# Autodesk Inventor assembly: Funnel Right
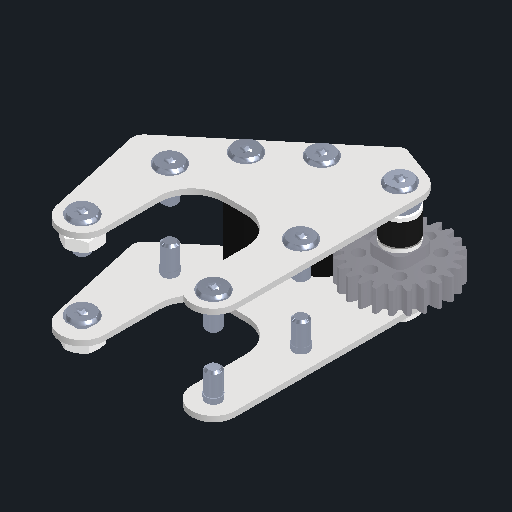
[picture p0: Inventor's stored thumbnail of the model, 512x512]
Saved by Autodesk Inventor 2025 (Build 290162000, 162)
## iProperties
Created: 2024-10-18
Part Number: Funnel Right
Document SubType Name: Assembly
Designer: Averey Ku
Author: averey
## Documents named in this file (19)
- D:\VEX\High Stakes\CAD\V2\Chassis\Drivebay Right\Funnel Right.iam
- D:\VEX\High Stakes\CAD\V2\Chassis\Drivebay Right\Funnel Gusset Right.ipt
- D:\VEX\High Stakes\CAD\ROBOPROS-CAD-Inventor\Motion\Spacers\Spacer Nylon .375 OD\NSpacer .375 OD x .500.ipt
- D:\VEX\High Stakes\CAD\ROBOPROS-CAD-Inventor\Motion\Spacers\Spacer Nylon .375 OD.ipt
- D:\VEX\High Stakes\CAD\ROBOPROS-CAD-Inventor\Structure\Hardware\Screw Steel - Star\SScrew Star Smooth 1.250.ipt
- D:\VEX\High Stakes\CAD\ROBOPROS-CAD-Inventor\Structure\Hardware\Screw Steel - Star.ipt
- D:\VEX\High Stakes\CAD\ROBOPROS-CAD-Inventor\Structure\Hardware\Nut Nylon\Nut Nylon - White.ipt
- D:\VEX\High Stakes\CAD\ROBOPROS-CAD-Inventor\Structure\Hardware\Nut Nylon.ipt
- D:\VEX\High Stakes\CAD\ROBOPROS-CAD-Inventor\Structure\Hardware\Screw Shoulder Robosource\SScrew Shoulder Smooth .375 x .12.ipt
- D:\VEX\High Stakes\CAD\ROBOPROS-CAD-Inventor\Structure\Hardware\Screw Shoulder Robosource.ipt
- D:\VEX\High Stakes\CAD\V2\Chassis\Drivebay Right\Half Cut HS 24T Gear, No Insert Right.ipt
- D:\VEX\High Stakes\CAD\V2\Chassis\Drivebay Right\Nut Keps Right1.ipt
- D:\vex_robotics_high_stakes\hardware\cad\VEX-CAD-Inventor\Motion\Spacers\Spacer Nylon .375 OD\NSpacer .375 OD x .250.ipt
- D:\vex_robotics_high_stakes\hardware\cad\VEX-CAD-Inventor\Motion\Spacers\Spacer Nylon .375 OD.ipt
- D:\vex_robotics_high_stakes\hardware\cad\VEX-CAD-Inventor\Motion\Spacers\Washer Teflon\TWasher .375 OD x .04000.ipt
- D:\vex_robotics_high_stakes\hardware\cad\VEX-CAD-Inventor\Motion\Spacers\Washer Teflon.ipt
- D:\vex_robotics_high_stakes\hardware\cad\VEX-CAD-Inventor\Motion\Spacers\Washer Steel\SWasher .375 OD x .015625.ipt
- D:\vex_robotics_high_stakes\hardware\cad\VEX-CAD-Inventor\Motion\Spacers\Washer Steel.ipt
- D:\VEX\High Stakes\CAD\ROBOPROS-CAD-Inventor\Structure\Hardware\Screw Shoulder Robosource\SScrew Shoulder Smooth .290 x .09.ipt
## Components (30 placed, 11 different names)
1. Funnel Gusset Right:1 — Mate:1, Insert:4, Insert:5, Insert:6, Insert:9, Insert:14, Insert:20, Insert:22, Insert:23
2. Funnel Gusset Right:2 — Mate:1, Insert:2, Insert:8, Insert:7, Insert:10, Insert:12, Insert:13, Insert:19, Insert:21
3. NSpacer .375 OD x .500:1 — Insert:1
4. NSpacer .375 OD x .500:2 — Insert:2, Insert:1
5. NSpacer .375 OD x .500:3 — Insert:4, Insert:3
6. NSpacer .375 OD x .500:4 — Insert:3
7. SScrew Star Smooth 1.250:1 — Insert:5
8. SScrew Star Smooth 1.250:2 — Insert:6
9. Nut Nylon - White:1 — Insert:8
10. Nut Nylon - White:2 — Insert:7
11. Nut Nylon - White:3 — Insert:12
12. Half Cut HS 24T Gear, No Insert Right:1 — Insert:13, Insert:18
13. Nut Keps Right1:1 — Insert:14
14. NSpacer .375 OD x .250:5 — Insert:15, Insert:16
15. TWasher .375 OD x .04000:1 — Insert:18, Insert:17
16. TWasher .375 OD x .04000:2 — Insert:15
17. SWasher .375 OD x .015625:1 — Insert:17, Insert:16
18. SScrew Star Smooth 1.250:3 — Insert:20
19. Nut Nylon - White:4 — Insert:19
20. SScrew Shoulder Smooth .290 x .09:3 — Insert:21
21. Nut Nylon - White:5 — Insert:22
22. SScrew Shoulder Smooth .290 x .09:4 — Insert:23
23. SScrew Shoulder Smooth .375 x .12:1 — Insert:9
24. SScrew Shoulder Smooth .375 x .12:5
25. SScrew Shoulder Smooth .375 x .12:6
26. SScrew Shoulder Smooth .375 x .12:7
27. SScrew Shoulder Smooth .375 x .12:2 — Insert:10
28. SScrew Shoulder Smooth .375 x .12:8
29. SScrew Shoulder Smooth .375 x .12:9
30. SScrew Shoulder Smooth .375 x .12:10
## Component patterns: (4 elements, first: SScrew Shoulder Smooth .375 x .12:1), (4 elements, first: SScrew Shoulder Smooth .375 x .12:2)
## Relationships (23: Insert 22, Mate 1)
- Mate:1: Funnel Gusset Right:1 ↔ Funnel Gusset Right:2
- Insert:2: Funnel Gusset Right:2 ↔ NSpacer .375 OD x .500:2
- Insert:1: NSpacer .375 OD x .500:1 ↔ NSpacer .375 OD x .500:2
- Insert:4: Funnel Gusset Right:1 ↔ NSpacer .375 OD x .500:3
- Insert:3: NSpacer .375 OD x .500:3 ↔ NSpacer .375 OD x .500:4
- Insert:5: Funnel Gusset Right:1 ↔ SScrew Star Smooth 1.250:1
- Insert:6: Funnel Gusset Right:1 ↔ SScrew Star Smooth 1.250:2
- Insert:8: Funnel Gusset Right:2 ↔ Nut Nylon - White:1
- Insert:7: Funnel Gusset Right:2 ↔ Nut Nylon - White:2
- Insert:9: Funnel Gusset Right:1 ↔ SScrew Shoulder Smooth .375 x .12:1
- Insert:10: Funnel Gusset Right:2 ↔ SScrew Shoulder Smooth .375 x .12:2
- Insert:12: Funnel Gusset Right:2 ↔ Nut Nylon - White:3
- Insert:13: Funnel Gusset Right:2 ↔ Half Cut HS 24T Gear, No Insert Right:1
- Insert:14: Funnel Gusset Right:1 ↔ Nut Keps Right1:1
- Insert:18: Half Cut HS 24T Gear, No Insert Right:1 ↔ TWasher .375 OD x .04000:1
- Insert:15: NSpacer .375 OD x .250:5 ↔ TWasher .375 OD x .04000:2
- Insert:17: TWasher .375 OD x .04000:1 ↔ SWasher .375 OD x .015625:1
- Insert:16: NSpacer .375 OD x .250:5 ↔ SWasher .375 OD x .015625:1
- Insert:20: Funnel Gusset Right:1 ↔ SScrew Star Smooth 1.250:3
- Insert:19: Funnel Gusset Right:2 ↔ Nut Nylon - White:4
- Insert:21 (1.5875 mm): Funnel Gusset Right:2 ↔ SScrew Shoulder Smooth .290 x .09:3
- Insert:22 (1.5875 mm): Funnel Gusset Right:1 ↔ Nut Nylon - White:5
- Insert:23: Funnel Gusset Right:1 ↔ SScrew Shoulder Smooth .290 x .09:4
